# Autodesk Inventor assembly: SPRZĘGŁO ZĘBATE MP
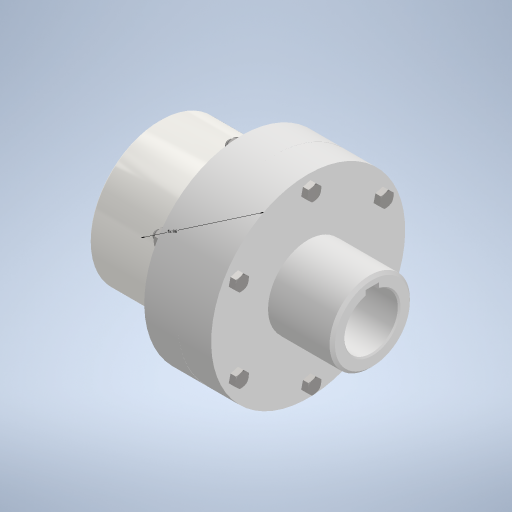
[picture p0: Inventor's stored thumbnail of the model, 512x512]
Saved by Autodesk Inventor 2024 (Build 280153000, 153)
## iProperties
Created: 2023-11-21
Part Number: SPRZĘGŁO ZĘBATE MP
Document SubType Name: Assembly
Designer: Wojciech
Author: Wojciech
## Documents named in this file (9)
- E:\studia\5sem\5sem1\PKM\PKMProjekt2MP2324\MarcinPrabuckiPROJEKT2SPRZĘGŁOZĘBATE\MarcinPrabuckiPROJEKT2SPRZĘGŁOZĘBATEsprawdzone\SPRZĘGŁOzłożenie\SPRZĘGŁO ZĘBATE MP.iam
- E:\studia\5sem\5sem1\PKM\PKMProjekt2MP2324\MarcinPrabuckiPROJEKT2SPRZĘGŁOZĘBATE\MarcinPrabuckiPROJEKT2SPRZĘGŁOZĘBATEsprawdzone\SPRZĘGŁOzłożenie\koło zębate.ipt
- E:\studia\5sem\5sem1\PKM\PKMProjekt2MP2324\MarcinPrabuckiPROJEKT2SPRZĘGŁOZĘBATE\MarcinPrabuckiPROJEKT2SPRZĘGŁOZĘBATEsprawdzone\SPRZĘGŁOzłożenie\Część5.ipt
- E:\studia\5sem\5sem1\PKM\PKMProjekt2MP2324\MarcinPrabuckiPROJEKT2SPRZĘGŁOZĘBATE\MarcinPrabuckiPROJEKT2SPRZĘGŁOZĘBATEsprawdzone\SPRZĘGŁOzłożenie\Część6.ipt
- E:\studia\5sem\5sem1\PKM\PKMProjekt2MP2324\MarcinPrabuckiPROJEKT2SPRZĘGŁOZĘBATE\MarcinPrabuckiPROJEKT2SPRZĘGŁOZĘBATEsprawdzone\SPRZĘGŁOzłożenie\Część7.ipt
- E:\studia\5sem\5sem1\PKM\PKMProjekt2MP2324\MarcinPrabuckiPROJEKT2SPRZĘGŁOZĘBATE\MarcinPrabuckiPROJEKT2SPRZĘGŁOZĘBATEsprawdzone\SPRZĘGŁOzłożenie\ANSI B18.2.3.5M - M6 x 1 x 60.ipt
- E:\studia\5sem\5sem1\PKM\PKMProjekt2MP2324\MarcinPrabuckiPROJEKT2SPRZĘGŁOZĘBATE\MarcinPrabuckiPROJEKT2SPRZĘGŁOZĘBATEsprawdzone\SPRZĘGŁOzłożenie\ANSI B18.22M - 6 N.ipt
- E:\studia\5sem\5sem1\PKM\PKMProjekt2MP2324\MarcinPrabuckiPROJEKT2SPRZĘGŁOZĘBATE\MarcinPrabuckiPROJEKT2SPRZĘGŁOZĘBATEsprawdzone\SPRZĘGŁOzłożenie\ANSI B18.2.2 - 12 - 24(06).ipt
- E:\studia\5sem\5sem1\PKM\PKMProjekt2MP2324\MarcinPrabuckiPROJEKT2SPRZĘGŁOZĘBATE\MarcinPrabuckiPROJEKT2SPRZĘGŁOZĘBATEsprawdzone\SPRZĘGŁOzłożenie\SPRZĘGŁO ZĘBATE MP\Design Accelerator\Spur Gears3.iam
## Components (24 placed, 8 different names)
1. koło zębate:1 — Równoległe:11, Zestawiające:4, Zestawiające:5
2. Część5:1 — Równoległe:7, Równoległe:8, Wstawiające:1, Wstawiające:2, Wstawiające:3, Wstawiające:4, Wstawiające:5, Wstawiające:6
3. Część6:1 — Równoległe:7, Równoległe:8, Równoległe:9, Równoległe:10, Obrotowe:1
4. Część7:1 — Równoległe:9, Równoległe:10
5. Podkładka okrągła (Metryczny) 6 N:1 — Wstawiające:1, Zestawiające:3
6. Podkładka okrągła (Metryczny) 6 N:2 — Wstawiające:2
7. Podkładka okrągła (Metryczny) 6 N:3 — Wstawiające:3
8. Podkładka okrągła (Metryczny) 6 N:4 — Wstawiające:4
9. Podkładka okrągła (Metryczny) 6 N:5 — Wstawiające:5
10. Podkładka okrągła (Metryczny) 6 N:6 — Wstawiające:6
11. Nakrętka sześciokątna - Calowy 12 - 24:1 — Zestawiające:1
12. Spur Gears:1 [sub-assembly] — Zestawiające:4, Zestawiające:5
13. ANSI B18.2.3.5M - M6 x 1 x 60:1 — Obrotowe:1
14. ANSI B18.2.3.5M - M6 x 1 x 60:2
15. ANSI B18.2.3.5M - M6 x 1 x 60:3
16. ANSI B18.2.3.5M - M6 x 1 x 60:4
17. ANSI B18.2.3.5M - M6 x 1 x 60:5
18. ANSI B18.2.3.5M - M6 x 1 x 60:6 — Zestawiające:1, Zestawiające:2
19. Nakrętka sześciokątna - Calowy 12 - 24:7 — Zestawiające:2, Zestawiające:3
20. Nakrętka sześciokątna - Calowy 12 - 24:8
21. Nakrętka sześciokątna - Calowy 12 - 24:9
22. Nakrętka sześciokątna - Calowy 12 - 24:10
23. Nakrętka sześciokątna - Calowy 12 - 24:11
24. Nakrętka sześciokątna - Calowy 12 - 24:12
## Component patterns: (6 elements, first: ANSI B18.2.3.5M - M6 x 1 x 60:1), (6 elements, first: Nakrętka sześciokątna - Calowy 12 - 24:7)
## Relationships (17: Insert 6, Flush 5, Mate 5, RevoluteJoint 1)
- Równoległe:7 [Flush]: Część5:1 ↔ Część6:1
- Równoległe:8 [Flush]: Część5:1 ↔ Część6:1
- Równoległe:9 [Flush]: Część6:1 ↔ Część7:1
- Równoległe:10 [Flush]: Część6:1 ↔ Część7:1
- Obrotowe:1 [RevoluteJoint]: Część6:1 ↔ ANSI B18.2.3.5M - M6 x 1 x 60:1
- Wstawiające:1 [Insert]: Część5:1 ↔ Podkładka okrągła (Metryczny) 6 N:1
- Wstawiające:2 [Insert]: Część5:1 ↔ Podkładka okrągła (Metryczny) 6 N:2
- Wstawiające:3 [Insert]: Część5:1 ↔ Podkładka okrągła (Metryczny) 6 N:3
- Wstawiające:4 [Insert]: Część5:1 ↔ Podkładka okrągła (Metryczny) 6 N:4
- Wstawiające:5 [Insert]: Część5:1 ↔ Podkładka okrągła (Metryczny) 6 N:5
- Wstawiające:6 [Insert]: Część5:1 ↔ Podkładka okrągła (Metryczny) 6 N:6
- Zestawiające:1 [Mate]: Nakrętka sześciokątna - Calowy 12 - 24:1 ↔ ANSI B18.2.3.5M - M6 x 1 x 60:6
- Zestawiające:2 [Mate]: ANSI B18.2.3.5M - M6 x 1 x 60:6 ↔ Nakrętka sześciokątna - Calowy 12 - 24:7
- Zestawiające:3 [Mate]: Podkładka okrągła (Metryczny) 6 N:1 ↔ Nakrętka sześciokątna - Calowy 12 - 24:7
- Równoległe:11 [Flush]: koło zębate:1
- Zestawiające:4 [Mate]: koło zębate:1 ↔ Spur Gears:1
- Zestawiające:5 [Mate]: koło zębate:1 ↔ Spur Gears:1
